# Autodesk Inventor assembly: Assemby 3
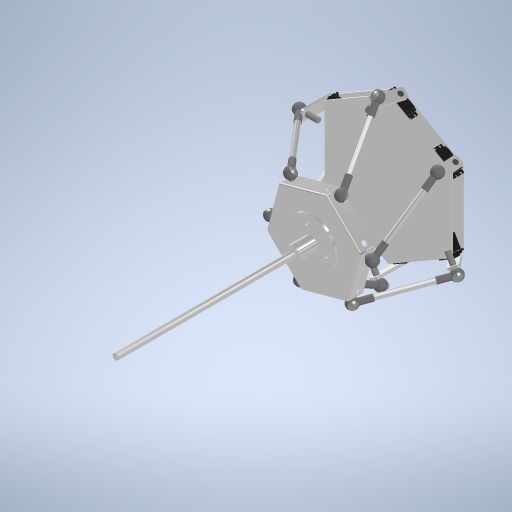
[picture p0: Inventor's stored thumbnail of the model, 512x512]
Saved by Autodesk Inventor 2023 (Build 270158000, 158)
## iProperties
Created: 2022-06-30
Part Number: Assemby 3
Document SubType Name: Assembly
Designer: earls
Mass: 2558.63 g
Surface Area: 5213.51 cm^2
Volume: 756.975 cm^3
Density: 3.38008 g/cm^3
Author: earls
## Documents named in this file (32)
- C:\Users\earls\Documents\stewart-platform\CAD\Assemby 3.iam
- C:\Users\earls\Documents\stewart-platform\CAD\Stewart Assembly.iam
- C:\Users\earls\Documents\stewart-platform\CAD\Moving platform.ipt
- C:\Users\earls\Documents\stewart-platform\CAD\Spherical joint\Part2.ipt
- C:\Users\earls\Documents\stewart-platform\CAD\Spherical joint\Part1.ipt
- C:\Users\earls\Documents\stewart-platform\CAD\Rod qty-6.ipt
- C:\Users\earls\Documents\stewart-platform\CAD\Test flange.ipt
- C:\Users\earls\Documents\stewart-platform\CAD\Strut.ipt
- C:\Users\earls\Documents\stewart-platform\CAD\Assemby 3\AIP\FEA\e0vycbpeo.fins
- C:\Users\earls\Documents\stewart-platform\CAD\Assemby 3\AIP\FEA\e0vycbq8w.fsat
- C:\Users\earls\Documents\stewart-platform\CAD\Assemby 3\AIP\FEA\e0vycbq9s.ftes
- C:\Users\earls\Documents\stewart-platform\CAD\Assemby 3\AIP\FEA\e0vycbq9s.fwiz
- C:\Users\earls\Documents\stewart-platform\CAD\Assemby 3\AIP\FEA\e0vycbq9t.fins
- C:\Users\earls\Documents\stewart-platform\CAD\Assemby 3\AIP\FEA\e0vycbqm8.fsat
- C:\Users\earls\Documents\stewart-platform\CAD\Assemby 3\AIP\FEA\e0vycbqn4.ftes
- C:\Users\earls\Documents\stewart-platform\CAD\Assemby 3\AIP\FEA\e0vycbqn4.fwiz
- C:\Users\earls\Documents\stewart-platform\CAD\Assemby 3\AIP\FEA\e0vycbqn5.fins
- C:\Users\earls\Documents\stewart-platform\CAD\Assemby 3\AIP\FEA\e0vycbqn5.fsat
- C:\Users\earls\Documents\stewart-platform\CAD\Assemby 3\AIP\FEA\e0vycbqu8.ftes
- C:\Users\earls\Documents\stewart-platform\CAD\Assemby 3\AIP\FEA\e0vycbqu8.fwiz
- C:\Users\earls\Documents\stewart-platform\CAD\Assemby 3\AIP\FEA\e0vycbts0.fmsh
- C:\Users\earls\Documents\stewart-platform\CAD\Assemby 3\AIP\FEA\e0vycbu74.fres
- C:\Users\earls\Documents\stewart-platform\CAD\Assemby 3\AIP\FEA\e0vycbyw0.fmsh
- C:\Users\earls\Documents\stewart-platform\CAD\Assemby 3\AIP\FEA\e0vycbz40.fres
- C:\Users\earls\Documents\stewart-platform\CAD\Assemby 3\AIP\FEA\e0vycc1uo.fmsh
- C:\Users\earls\Documents\stewart-platform\CAD\Assemby 3\AIP\FEA\e0vycc1vk.fres
- C:\Users\earls\Documents\stewart-platform\CAD\Assemby 3\AIP\FEA\e0vycc3uo.fmsh
- C:\Users\earls\Documents\stewart-platform\CAD\Assemby 3\AIP\FEA\e0vycc3up.fres
- C:\Users\earls\Documents\stewart-platform\CAD\Assemby 3\AIP\FEA\e0vycc7eo.fmsh
- C:\Users\earls\Documents\stewart-platform\CAD\Assemby 3\AIP\FEA\e0vycc7ep.fres
- C:\Users\earls\Documents\stewart-platform\CAD\Assemby 3\AIP\FEA\e0vycc8hs.fmsh
- C:\Users\earls\Documents\stewart-platform\CAD\Assemby 3\AIP\FEA\e0vycc8ht.fres
## Components (34 placed, 7 different names)
1. Stewart Assembly:1 [sub-assembly] — Insert:1, Insert:4, Insert:5, Insert:7, Insert:10, Insert:12, Mate:28
2. Moving platform:1 — Insert:2, Insert:3, Insert:6, Insert:8, Insert:9, Insert:11, Mate:28, Mate:29, Mate:30, Mate:31, Mate:32, Mate:33
3. Part2:1 — Insert:2, Ball:1
4. Part2:2 — Insert:1, Ball:2
5. Part1:1 — Ball:2, Mate:3, Mate:4
6. Part1:2 — Ball:1, Mate:5, Mate:6
7. Rod qty-6:1 — Mate:3, Mate:4, Mate:5, Mate:6
8. Rod qty-6:2 — Mate:7, Mate:8, Mate:9
9. Part1:3 — Ball:3, Mate:9
10. Part2:3 — Insert:3, Ball:3
11. Part2:4 — Insert:4, Ball:4
12. Part1:4 — Ball:4, Mate:7, Mate:8
13. Part1:5 — Ball:5, Mate:10, Mate:11
14. Part2:5 — Insert:5, Ball:5
15. Part1:6 — Ball:6, Mate:12, Mate:13
16. Part2:6 — Insert:6, Ball:6
17. Rod qty-6:3 — Mate:10, Mate:11, Mate:12, Mate:13
18. Part1:7 — Ball:8, Mate:16, Mate:24
19. Part2:7 — Insert:8, Ball:8
20. Part1:8 — Ball:7, Mate:14, Mate:15
21. Part2:8 — Insert:7, Ball:7
22. Rod qty-6:4 — Mate:14, Mate:15, Mate:16, Mate:24
23. Part1:9 — Ball:9, Mate:18, Mate:19
24. Part2:9 — Insert:9, Ball:9
25. Part1:10 — Ball:10, Mate:17, Mate:23
26. Part2:10 — Insert:10, Ball:10
27. Rod qty-6:5 — Mate:17, Mate:18, Mate:19, Mate:23
28. Part1:11 — Ball:11, Mate:21, Mate:22
29. Part2:11 — Insert:11, Ball:11
30. Part1:12 — Ball:12, Mate:20
31. Part2:12 — Insert:12, Ball:12
32. Rod qty-6:6 — Mate:20, Mate:21, Mate:22
33. Test flange:1 — Mate:29, Mate:30, Mate:31, Mate:32, Mate:33, Rigid:1
34. Strut:1 — Rigid:1
## Relationships (53: Mate 28, Insert 12, BallJoint 12, WeldJoint 1)
- Insert:1 (-3 mm): Stewart Assembly:1 ↔ Part2:2
- Insert:2 (-3 mm): Moving platform:1 ↔ Part2:1
- Ball:1: Part2:1 ↔ Part1:2
- Ball:2: Part2:2 ↔ Part1:1
- Mate:3: Part1:1 ↔ Rod qty-6:1
- Mate:4: Part1:1 ↔ Rod qty-6:1
- Mate:5: Part1:2 ↔ Rod qty-6:1
- Mate:6: Part1:2 ↔ Rod qty-6:1
- Insert:3 (-3 mm): Moving platform:1 ↔ Part2:3
- Ball:3: Part1:3 ↔ Part2:3
- Insert:4 (-3 mm): Stewart Assembly:1 ↔ Part2:4
- Ball:4: Part2:4 ↔ Part1:4
- Mate:7: Rod qty-6:2 ↔ Part1:4
- Mate:8: Rod qty-6:2 ↔ Part1:4
- Mate:9: Rod qty-6:2 ↔ Part1:3
- Insert:5 (-3 mm): Stewart Assembly:1 ↔ Part2:5
- Insert:6 (-3 mm): Moving platform:1 ↔ Part2:6
- Ball:5: Part1:5 ↔ Part2:5
- Ball:6: Part1:6 ↔ Part2:6
- Mate:10: Part1:5 ↔ Rod qty-6:3
- Mate:11: Part1:5 ↔ Rod qty-6:3
- Mate:12: Part1:6 ↔ Rod qty-6:3
- Mate:13: Part1:6 ↔ Rod qty-6:3
- Insert:7 (-3 mm): Stewart Assembly:1 ↔ Part2:8
- Insert:8 (-3 mm): Moving platform:1 ↔ Part2:7
- Ball:7: Part1:8 ↔ Part2:8
- Ball:8: Part1:7 ↔ Part2:7
- Mate:14: Part1:8 ↔ Rod qty-6:4
- Mate:15: Part1:8 ↔ Rod qty-6:4
- Mate:16: Part1:7 ↔ Rod qty-6:4
- Insert:9 (-3 mm): Moving platform:1 ↔ Part2:9
- Ball:9: Part1:9 ↔ Part2:9
- Insert:10 (-3 mm): Stewart Assembly:1 ↔ Part2:10
- Ball:10: Part1:10 ↔ Part2:10
- Mate:17: Part1:10 ↔ Rod qty-6:5
- Mate:18: Part1:9 ↔ Rod qty-6:5
- Mate:19: Part1:9 ↔ Rod qty-6:5
- Insert:11 (-3 mm): Moving platform:1 ↔ Part2:11
- Insert:12 (-3 mm): Stewart Assembly:1 ↔ Part2:12
- Ball:11: Part1:11 ↔ Part2:11
- Ball:12: Part1:12 ↔ Part2:12
- Mate:20: Part1:12 ↔ Rod qty-6:6
- Mate:21: Part1:11 ↔ Rod qty-6:6
- Mate:22: Part1:11 ↔ Rod qty-6:6
- Mate:23: Part1:10 ↔ Rod qty-6:5
- Mate:24: Part1:7 ↔ Rod qty-6:4
- Mate:28 (168.085 mm): Stewart Assembly:1 ↔ Moving platform:1
- Mate:29: Moving platform:1 ↔ Test flange:1
- Mate:30: Moving platform:1 ↔ Test flange:1
- Mate:31: Moving platform:1 ↔ Test flange:1
- Mate:32: Moving platform:1 ↔ Test flange:1
- Mate:33: Moving platform:1 ↔ Test flange:1
- Rigid:1 [WeldJoint]: Test flange:1 ↔ Strut:1
## Named parameters: sa_6 = 2000, sa_0 = 100, sa_1 = 4000, sa_2 = 200, sa_3 = 15000, sa_4 = 18000, sa_5 = 23000, sa_7 = 27000
note: some values were not read from the file. Shown as the stored number, unit unknown: "sa_6", "sa_0", "sa_1", "sa_2", "sa_3", "sa_4", "sa_5", "sa_7".
